# Autodesk Inventor assembly: Сборка1
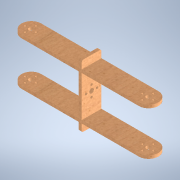
[picture p0: Inventor's stored thumbnail of the model, 180x180]
Saved by Autodesk Inventor 2020.1 (Build 241239000, 239)
## iProperties
Created: 2021-08-12
Part Number: Сборка1
Document SubType Name: Assembly
Designer: Ni3na
Author: Ni3na
## Documents named in this file (3)
- D:\GitHub\avatar-kvantoriada\3D\Сборка1.iam
- D:\GitHub\avatar-kvantoriada\3D\Деталь1.ipt
- D:\GitHub\avatar-kvantoriada\3D\Деталь2.ipt
## Components (3 placed, 2 different names)
1. Деталь1:1 — Жесткий:2
2. Деталь1:2 — Жесткий:1
3. Деталь2:1 — Жесткий:1, Жесткий:2
## Relationships (2: WeldJoint 2)
- Жесткий:1 [WeldJoint]: Деталь1:2 ↔ Деталь2:1
- Жесткий:2 [WeldJoint]: Деталь1:1 ↔ Деталь2:1
